# Autodesk Inventor assembly: 4_Camera
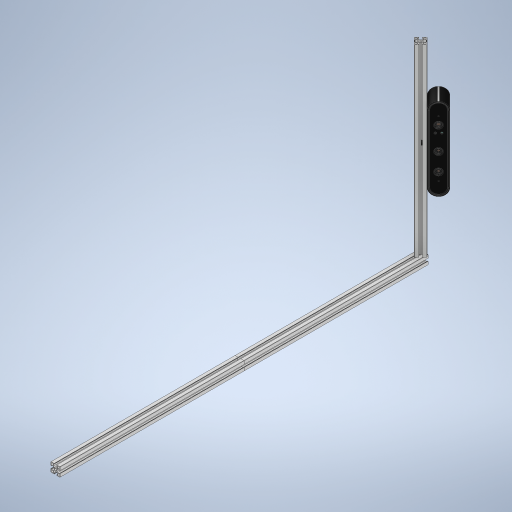
[picture p0: Inventor's stored thumbnail of the model, 512x512]
Saved by Autodesk Inventor 2024 (Build 280153000, 153)
## iProperties
Created: 2023-11-26
Part Number: 4_Camera
Document SubType Name: Assembly
Designer: 박동준
Author: 박동준
## Documents named in this file (3)
- C:\Users\박동준\OneDrive - 연세대학교 (Yonsei University)\바탕 화면\박동준\대학생할\로봇\Humanoid\7축 매니퓰레이터\하드웨어\rh_plus_7_axis_robot_arm_hardware\Assembly\4_Camera.iam
- C:\Users\박동준\OneDrive - 연세대학교 (Yonsei University)\바탕 화면\박동준\대학생할\로봇\Humanoid\7축 매니퓰레이터\하드웨어\rh_plus_7_axis_robot_arm_hardware\Part\Other Parts\Astra_depth_camera.ipt
- C:\Users\박동준\OneDrive - 연세대학교 (Yonsei University)\바탕 화면\박동준\대학생할\로봇\Humanoid\7축 매니퓰레이터\하드웨어\rh_plus_7_axis_robot_arm_hardware\Part\Other Parts\Aluminum_Profile_2020.ipt
## Components (4 placed, 2 different names)
1. Astra_depth_camera:1 — Mate:4, Flush:3, Flush:4
2. Aluminum_Profile_2020:1 — Mate:1, Flush:1, Flush:2
3. Aluminum_Profile_2020:2 — Mate:1, Flush:1, Flush:2, Mate:2, Angle:1, Mate:3
4. Aluminum_Profile_2020:3 — Mate:2, Angle:1, Mate:3, Mate:4, Flush:3, Flush:4
## Relationships (9: Mate 4, Flush 4, Angle 1)
- Mate:1: Aluminum_Profile_2020:1 ↔ Aluminum_Profile_2020:2
- Flush:1: Aluminum_Profile_2020:1 ↔ Aluminum_Profile_2020:2
- Flush:2: Aluminum_Profile_2020:1 ↔ Aluminum_Profile_2020:2
- Mate:2: Aluminum_Profile_2020:2 ↔ Aluminum_Profile_2020:3
- Angle:1 (45 deg): Aluminum_Profile_2020:2 ↔ Aluminum_Profile_2020:3
- Mate:3: Aluminum_Profile_2020:2 ↔ Aluminum_Profile_2020:3
- Mate:4: Astra_depth_camera:1 ↔ Aluminum_Profile_2020:3
- Flush:3 (-10 mm): Astra_depth_camera:1 ↔ Aluminum_Profile_2020:3
- Flush:4 (100 mm): Astra_depth_camera:1 ↔ Aluminum_Profile_2020:3
